# Autodesk Inventor assembly: gripper
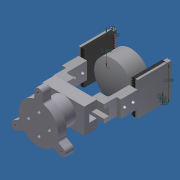
[picture p0: Inventor's stored thumbnail of the model, 180x180]
Saved by Autodesk Inventor 2012 (Build 160160000, 160)
## iProperties
Created: 2012-07-09
Part Number: gripper
Document SubType Name: Assembly
Designer: Ed
Author: Ed
## Documents named in this file (8)
- C:\Users\Ed\Documents\masters\CAD\Gripper\gripper.iam
- C:\Users\Ed\Documents\masters\CAD\Gripper\gripper plate.ipt
- C:\Users\Ed\Documents\masters\CAD\Gripper\gripper.ipt
- C:\Users\Ed\Documents\masters\CAD\Gripper\IRB120 plate.ipt
- C:\Users\Ed\Documents\masters\CAD\Gripper\gripper jaw.ipt
- C:\Users\Ed\Documents\masters\CAD\objects\door knob.ipt
- C:\Users\Ed\Documents\masters\CAD\Gripper\gripper jaw extension.ipt
- C:\Users\Ed\Documents\masters\CAD\Gripper\gripper pad.ipt
## Components (10 placed, 7 different names)
1. gripper plate:1 — Insert:1, Insert:2, Insert:3, Insert:4
2. gripper:1 — Insert:1, Insert:4, Flush:3, Flush:4, Mate:2
3. IRB120 plate:1 — Insert:2, Insert:3
4. gripper jaw:1 — Flush:1, Flush:2, Flush:4, Gripper Position, Insert:5, Insert:6
5. gripper jaw:2 — Flush:1, Flush:2, Flush:3, Gripper Position, Insert:7, Insert:8
6. door knob:1 — Mate:2
7. gripper jaw extension:1 — Mate:4, Flush:6, Flush:7, Insert:7, Insert:8
8. gripper pad:1 — Mate:4, Flush:6, Flush:7
9. gripper jaw extension:2 — Mate:3, Flush:5, Flush:8, Insert:5, Insert:6
10. gripper pad:2 — Mate:3, Flush:5, Flush:8
## Relationships (20: Insert 8, Flush 8, Mate 4)
- Insert:1: gripper plate:1 ↔ gripper:1
- Insert:2: gripper plate:1 ↔ IRB120 plate:1
- Insert:3: gripper plate:1 ↔ IRB120 plate:1
- Insert:4: gripper plate:1 ↔ gripper:1
- Flush:1: gripper jaw:1 ↔ gripper jaw:2
- Flush:2: gripper jaw:1 ↔ gripper jaw:2
- Flush:3 (-49.1744 mm): gripper:1 ↔ gripper jaw:2
- Flush:4: gripper:1 ↔ gripper jaw:1
- Gripper Position [Mate] (-76.2 mm): gripper jaw:1 ↔ gripper jaw:2
- Mate:2: gripper:1 ↔ door knob:1
- Mate:3: gripper jaw extension:2 ↔ gripper pad:2
- Mate:4: gripper jaw extension:1 ↔ gripper pad:1
- Flush:5: gripper jaw extension:2 ↔ gripper pad:2
- Flush:6: gripper jaw extension:1 ↔ gripper pad:1
- Flush:7: gripper jaw extension:1 ↔ gripper pad:1
- Flush:8: gripper jaw extension:2 ↔ gripper pad:2
- Insert:5: gripper jaw:1 ↔ gripper jaw extension:2
- Insert:6: gripper jaw:1 ↔ gripper jaw extension:2
- Insert:7: gripper jaw:2 ↔ gripper jaw extension:1
- Insert:8: gripper jaw:2 ↔ gripper jaw extension:1
